# Autodesk Inventor assembly: A_MiniDrone
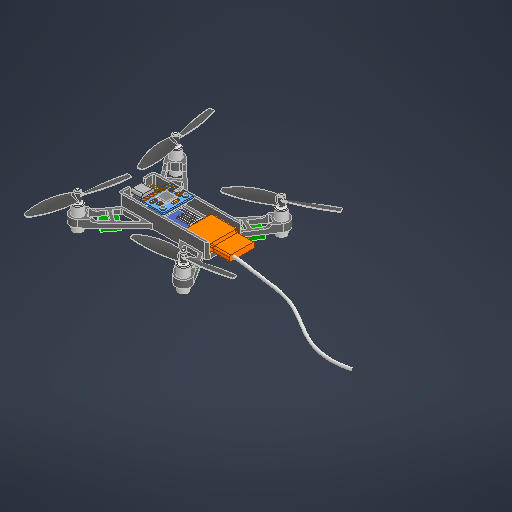
[picture p0: Inventor's stored thumbnail of the model, 512x512]
Saved by Autodesk Inventor 2026 (Build 300175000, 175)
## iProperties
Created: 2025-08-01
Part Number: A_MiniDrone
Document SubType Name: Assembly
Designer: FAL
Author: FAL
## Documents named in this file (9)
- C:\Users\FAL\Projekte\local\MiniDrone\Hardware\CAD\A_MiniDrone.iam
- C:\Users\FAL\Projekte\local\MiniDrone\Hardware\CAD\P_DroneCase.ipt
- C:\Users\FAL\Projekte\local\MiniDrone\Hardware\CAD\extern\ESP32-C3 supermini v5\ESP32-C3 supermini v5\ESP32-C3 supermini v5.iam
- C:\Users\FAL\Projekte\local\MiniDrone\Hardware\CAD\extern\MPU6050 v2\MPU6050 v2\MPU6050 v2.ipt
- C:\Users\FAL\Projekte\local\MiniDrone\Hardware\CAD\P_Akku_1S.ipt
- C:\Users\FAL\Projekte\local\MiniDrone\Hardware\CAD\P_Motor.ipt
- C:\Users\FAL\Projekte\local\MiniDrone\Hardware\CAD\P_Motordriver.ipt
- C:\Users\FAL\Projekte\local\MiniDrone\Hardware\CAD\P_Prop.ipt
- C:\Users\FAL\Projekte\local\MiniDrone\Hardware\CAD\P_R6DSM.ipt
## Components (17 placed, 8 different names)
1. P_DroneCase:1 — Passend:1, Passend:2, Fluchtend:1, Passend:3, Passend:4, Passend:5, Passend:6, Passend:12, Passend:13, Passend:14, Passend:15, Passend:16, Passend:17, Passend:18
2. ESP32-C3 supermini v5:1 [sub-assembly]
3. MPU6050 v2:1 — Passend:12, Passend:13
4. P_Akku_1S:1
5. P_Motor:1 — Passend:3, Fluchtend:3, Passend:8
6. P_Motor:2 — Passend:4, Fluchtend:3, Fluchtend:4, Fluchtend:5, Passend:7
7. P_Motor:3 — Passend:5, Fluchtend:5, Passend:9, Passend:11, Passend:18
8. P_Motor:4 — Passend:6, Fluchtend:4, Passend:10
9. P_Motordriver:1 — Passend:16
10. P_Motordriver:2 — Passend:15
11. P_Motordriver:3 — Passend:14
12. P_Motordriver:4 — Passend:17
13. P_Prop:1 — Passend:7, Fluchtend:6
14. P_Prop:2 — Passend:8, Fluchtend:6, Fluchtend:7
15. P_Prop:3 — Passend:10, Fluchtend:7, Fluchtend:8
16. P_Prop:4 — Passend:9, Fluchtend:8, Passend:11
17. P_R6DSM:1
## Relationships (25: Mate 18, Flush 7)
- Passend:1 [Mate]: P_DroneCase:1
- Passend:2 [Mate]: P_DroneCase:1
- Fluchtend:1 [Flush]: P_DroneCase:1
- Passend:3 [Mate]: P_DroneCase:1 ↔ P_Motor:1
- Passend:4 [Mate]: P_DroneCase:1 ↔ P_Motor:2
- Passend:5 [Mate]: P_DroneCase:1 ↔ P_Motor:3
- Passend:6 [Mate]: P_DroneCase:1 ↔ P_Motor:4
- Fluchtend:3 [Flush]: P_Motor:1 ↔ P_Motor:2
- Fluchtend:4 [Flush]: P_Motor:2 ↔ P_Motor:4
- Fluchtend:5 [Flush]: P_Motor:2 ↔ P_Motor:3
- Passend:7 [Mate]: P_Motor:2 ↔ P_Prop:1
- Passend:8 [Mate]: P_Motor:1 ↔ P_Prop:2
- Passend:9 [Mate]: P_Motor:3 ↔ P_Prop:4
- Passend:10 [Mate]: P_Motor:4 ↔ P_Prop:3
- Fluchtend:6 [Flush]: P_Prop:1 ↔ P_Prop:2
- Fluchtend:7 [Flush]: P_Prop:2 ↔ P_Prop:3
- Fluchtend:8 [Flush]: P_Prop:3 ↔ P_Prop:4
- Passend:11 [Mate] (1 mm): P_Motor:3 ↔ P_Prop:4
- Passend:12 [Mate]: P_DroneCase:1 ↔ MPU6050 v2:1
- Passend:13 [Mate]: P_DroneCase:1 ↔ MPU6050 v2:1
- Passend:14 [Mate]: P_DroneCase:1 ↔ P_Motordriver:3
- Passend:15 [Mate]: P_DroneCase:1 ↔ P_Motordriver:2
- Passend:16 [Mate]: P_DroneCase:1 ↔ P_Motordriver:1
- Passend:17 [Mate]: P_DroneCase:1 ↔ P_Motordriver:4
- Passend:18 [Mate] (5 mm): P_DroneCase:1 ↔ P_Motor:3
